# Autodesk Inventor assembly: Belt Tensioner Assy
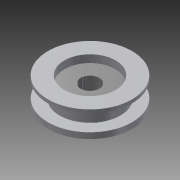
[picture p0: Inventor's stored thumbnail of the model, 180x180]
Saved by Autodesk Inventor 2015 SP1 (Build 190203100, 203)
## iProperties
Created: 2015-02-24
Part Number: Belt Tensioner Assy
Document SubType Name: Assembly
Designer: Andrew
Author: Andrew
## Documents named in this file (3)
- C:\Users\Andrew\Documents\model\Belt Tensioner Assy.iam
- C:\Users\Andrew\Documents\model\Bearing.ipt
- C:\Users\Andrew\Documents\model\Belt Tensioner.ipt
## Components (2 placed, 2 different names)
1. Bearing:1 — Mate:1, Mate:2
2. Belt Tensioner:1 — Mate:1, Mate:2, Flush:1, Flush:2, Flush:3
## Relationships (5: Flush 3, Mate 2)
- Mate:1: Bearing:1 ↔ Belt Tensioner:1
- Mate:2: Bearing:1 ↔ Belt Tensioner:1
- Flush:1: Belt Tensioner:1
- Flush:2: Belt Tensioner:1
- Flush:3: Belt Tensioner:1
